# Autodesk Inventor assembly: openmv4_h7
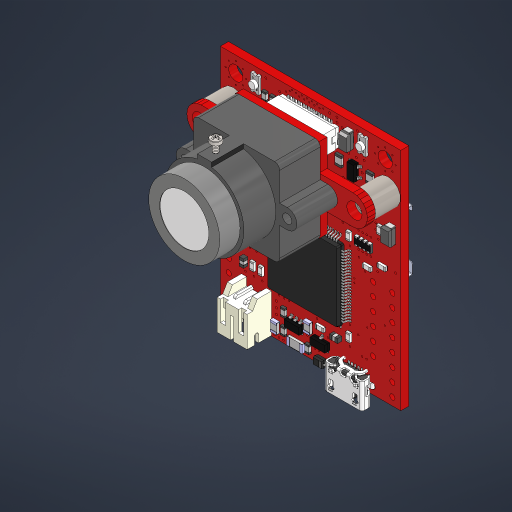
[picture p0: Inventor's stored thumbnail of the model, 512x512]
Saved by Autodesk Inventor 2024.2 (Build 282272000, 272)
## iProperties
Created: 2019-09-24
Part Number: openmv4_h7
Description: STEP AP214
Document SubType Name: Assembly
Designer: Hanaoka
Sending System: SolidWorks 2016
Preprocessor: SwSTEP 2.0
Title: openmv4_h7.STEP
Revision Number: ANY
## Documents named in this file (5)
- G:\共有ドライブ\reRo\05_個人\hanaoka\inventor\CameraUnit\OpenMV_H7\OpenMV_H7.iam
- G:\共有ドライブ\reRo\05_個人\hanaoka\inventor\CameraUnit\OpenMV_H7\openmv4_h7_base_® ã¬®«ç ­¨î.iam
- G:\共有ドライブ\reRo\05_個人\hanaoka\inventor\CameraUnit\OpenMV_H7\openmv4_ov7725_® ã¬®«ç ­¨î.iam
- G:\共有ドライブ\reRo\05_個人\hanaoka\inventor\CameraUnit\OpenMV_H7\LENS_Standard_® ã¬®«ç ­¨î.ipt
- G:\共有ドライブ\reRo\05_個人\hanaoka\inventor\CameraUnit\OpenMV_H7\pan head cross recess screw_iso_ISO 7045 - M1 x 4 - Z - 4S.ipt
## Components (4 placed, 4 different names)
1. openmv4_h7_base_® ã¬®«ç ­¨î_1 [sub-assembly]
2. openmv4_ov7725_® ã¬®«ç ­¨î_2 [sub-assembly] — 挿入:1
3. LENS_Standard_® ã¬®«ç ­¨î_6 — 挿入:1
4. pan head cross recess screw_iso_ISO 7045 - M1 x 4 - Z - 4S_9
## Relationships (1: Insert 1)
- 挿入:1 [Insert] (-4 mm): openmv4_ov7725_® ã¬®«ç ­¨î_2 ↔ LENS_Standard_® ã¬®«ç ­¨î_6
